# Autodesk Inventor assembly: Bar_connection_assembly
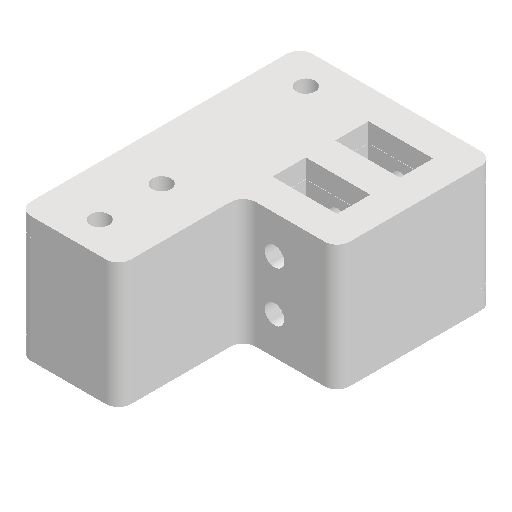
[picture p0: Inventor's stored thumbnail of the model, 512x512]
Saved by Autodesk Inventor 2022 (Build 260153000, 153)
## iProperties
Created: 2022-08-24
Part Number: Bar_connection_assembly
Document SubType Name: Assembly
Designer: dell
Mass: 26.483 g
Surface Area: 177.753 cm^2
Volume: 26.483 cm^3
Density: 1 g/cm^3
Author: dell
## Documents named in this file (3)
- D:\xxxx\Uni\Part IV\MECHENG_700\Part_IV_project_CAD\Bird_skeleton_prototypes\Wing_drone_V1\Bird_wing_V2\Wing_shoulder\Bar_connection_assembly.iam
- D:\xxxx\Uni\Part IV\MECHENG_700\Part_IV_project_CAD\Bird_skeleton_prototypes\Wing_drone_V1\Bird_wing_V2\Wing_shoulder\Bar_connection_plate.ipt
- D:\xxxx\Uni\Part IV\MECHENG_700\Part_IV_project_CAD\Bird_skeleton_prototypes\Wing_drone_V1\Bird_wing_V2\Wing_shoulder\Bar_connection_block.ipt
## Components (3 placed, 2 different names)
1. Bar_connection_plate:1
2. Bar_connection_block:1
3. Bar_connection_plate:2
## Relationships (6: Flush 4, Mate 2)
- [Mate]: Bar_connection_plate:1 ↔ Bar_connection_block:1
- [Flush]: Bar_connection_plate:1 ↔ Bar_connection_block:1
- [Flush]: Bar_connection_plate:1 ↔ Bar_connection_block:1
- [Mate]: Bar_connection_block:1 ↔ Bar_connection_plate:2
- [Flush]: Bar_connection_block:1 ↔ Bar_connection_plate:2
- [Flush]: Bar_connection_block:1 ↔ Bar_connection_plate:2
## Named parameters: d9_d15 = 0 mm, d10_d16 = 0 mm, d11_d17 = 0 mm
